# Autodesk Inventor assembly: Antrieb
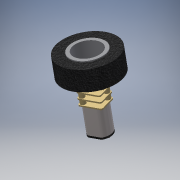
[picture p0: Inventor's stored thumbnail of the model, 180x180]
Saved by Autodesk Inventor 2017.3 (Build 213257000, 257)
## iProperties
Part Number: Antrieb
Material: Generisch
Document SubType Name: Assembly
Designer: Enno-LT
Author: Enno-LT
## Documents named in this file (4)
- C:\Users\Enno-LT\Documents\Inventor\Kugelprojekt\Antrieb.iam
- C:\Users\Enno-LT\Desktop\Kugel Projekt\Antriebsrad_V1.ipt
- C:\Users\Enno-LT\Documents\Inventor\Content Center Files\R2017\de-DE\AS 1427(10)\AS 1427 - M2 x 5(7).ipt
- C:\Users\Enno-LT\Desktop\Kugel Projekt\SPG10 Motor.ipt
## Components (3 placed, 3 different names)
1. Antriebsrad_V1:1 — Passend:1, Passend:2, Fluchtend:1, Winkel:1
2. AS 1427 (8) - Metrisch M2 x 5:1 — Passend:1, Passend:3, Winkel:1
3. SPG10 Motor:1 — Passend:2, Fluchtend:1, Passend:3
## Relationships (5: Mate 3, Flush 1, Angle 1)
- Passend:1 [Mate]: Antriebsrad_V1:1 ↔ AS 1427 (8) - Metrisch M2 x 5:1
- Passend:2 [Mate]: Antriebsrad_V1:1 ↔ SPG10 Motor:1
- Fluchtend:1 [Flush]: Antriebsrad_V1:1 ↔ SPG10 Motor:1
- Passend:3 [Mate]: AS 1427 (8) - Metrisch M2 x 5:1 ↔ SPG10 Motor:1
- Winkel:1 [Angle] (0 deg): Antriebsrad_V1:1 ↔ AS 1427 (8) - Metrisch M2 x 5:1
